# Autodesk Inventor assembly: Basket Assembly
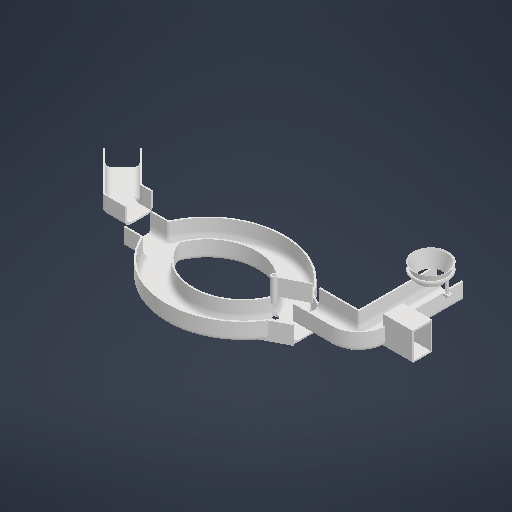
[picture p0: Inventor's stored thumbnail of the model, 512x512]
Saved by Autodesk Inventor 2026.2 (Build 302298010, 298A)
## iProperties
Created: 2026-03-21
Part Number: Basket Assembly
Document SubType Name: Assembly
Designer: Amir
Author: Amir
## Documents named in this file (8)
- F:\Semester 4\Basics of Mechatronics\Project\Basket Assembly.iam
- F:\Semester 4\Basics of Mechatronics\Project\path.ipt
- F:\Semester 4\Basics of Mechatronics\Project\basket holder.ipt
- F:\Semester 4\Basics of Mechatronics\Project\basket.ipt
- F:\Semester 4\Basics of Mechatronics\Project\Sorting.ipt
- F:\Semester 4\Basics of Mechatronics\Project\Path of Storage.ipt
- F:\Semester 4\Basics of Mechatronics\Project\Gate.ipt
- F:\Semester 4\Basics of Mechatronics\Project\Path from IR to PIN.ipt
## Components (7 placed, 7 different names)
1. Path:1 — Mate:1, Mate:2, Mate:4, Mate:5, Mate:6
2. basket holder:1 — Mate:1, Mate:2, Mate:3
3. basket:1 — Mate:3
4. Path from IR to PIN:1 — Mate:4, Mate:5, Mate:6, Mate:7, Mate:8
5. Sorting:1 — Mate:7, Mate:8, Mate:9, Mate:10, Mate:11, Mate:12, Mate:13
6. Gate:1 — Mate:9, Mate:10
7. Path of Storage:1 — Mate:11, Mate:12, Mate:13
## Relationships (13: Mate 13)
- Mate:1: Path:1 ↔ basket holder:1
- Mate:2: Path:1 ↔ basket holder:1
- Mate:3: basket holder:1 ↔ basket:1
- Mate:4: Path:1 ↔ Path from IR to PIN:1
- Mate:5: Path:1 ↔ Path from IR to PIN:1
- Mate:6: Path:1 ↔ Path from IR to PIN:1
- Mate:7: Path from IR to PIN:1 ↔ Sorting:1
- Mate:8: Path from IR to PIN:1 ↔ Sorting:1
- Mate:9: Sorting:1 ↔ Gate:1
- Mate:10: Sorting:1 ↔ Gate:1
- Mate:11: Sorting:1 ↔ Path of Storage:1
- Mate:12: Sorting:1 ↔ Path of Storage:1
- Mate:13: Sorting:1 ↔ Path of Storage:1
